# Autodesk Inventor assembly: _osmobuddy_top
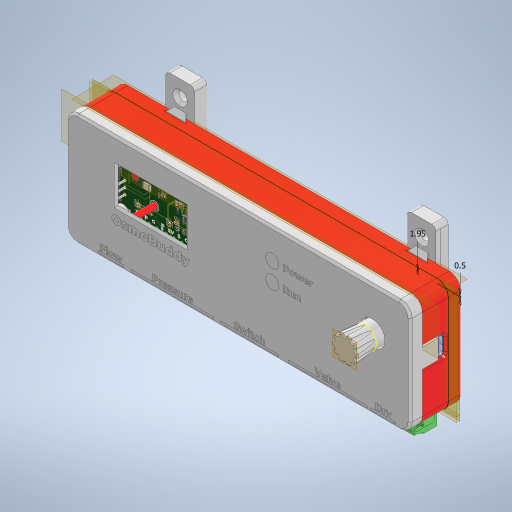
[picture p0: Inventor's stored thumbnail of the model, 512x512]
Saved by Autodesk Inventor 2024.3 (Build 283343000, 343)
## iProperties
Created: 2024-08-31
Part Number: _osmobuddy_top
Document SubType Name: Assembly
Designer: atrus
Author: atrus
## Documents named in this file (6)
- C:\Users\atrus\Dropbox\elec\Mechanical\osmoBuddy\_osmobuddy_top.iam
- C:\Users\atrus\Dropbox\elec\Mechanical\osmoBuddy\PCB\osmobuddy_v1.iam
- C:\Users\atrus\Dropbox\elec\Mechanical\osmoBuddy\osmobuddy_bottom.ipt
- C:\Users\atrus\Dropbox\elec\Mechanical\osmoBuddy\osmobuddy_top.ipt
- C:\Users\atrus\Dropbox\elec\Mechanical\osmoBuddy\_Wallmount.ipt
- C:\Users\atrus\Dropbox\elec\Mechanical\osmoBuddy\Knob.ipt
## Components (5 placed, 5 different names)
1. osmobuddy_v1:1 [sub-assembly] — Flush:1, Flush:2, Flush:3, Flush:4, Flush:9, Flush:10
2. osmobuddy_bottom:1 — Flush:1, Flush:2, Flush:3, Flush:4, Flush:5, Flush:6, Flush:7, Flush:8
3. osmobuddy_top:1 — Flush:5, Flush:6
4. _Wallmount:1 — Flush:7, Flush:8
5. Knob:1 — Flush:9, Flush:10
## Relationships (10: Flush 10)
- Flush:1: osmobuddy_v1:1 ↔ osmobuddy_bottom:1
- Flush:2: osmobuddy_v1:1 ↔ osmobuddy_bottom:1
- Flush:3 (0.2032 mm): osmobuddy_v1:1 ↔ osmobuddy_bottom:1
- Flush:4 (0.2032 mm): osmobuddy_v1:1 ↔ osmobuddy_bottom:1
- Flush:5: osmobuddy_bottom:1 ↔ osmobuddy_top:1
- Flush:6: osmobuddy_bottom:1 ↔ osmobuddy_top:1
- Flush:7: osmobuddy_bottom:1 ↔ _Wallmount:1
- Flush:8: osmobuddy_bottom:1 ↔ _Wallmount:1
- Flush:9: osmobuddy_v1:1 ↔ Knob:1
- Flush:10 (0.2032 mm): osmobuddy_v1:1 ↔ Knob:1
